# Autodesk Inventor assembly: BrImp_Assembly
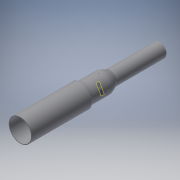
[picture p0: Inventor's stored thumbnail of the model, 180x180]
Saved by Autodesk Inventor 2018 (Build 220112000, 112)
## iProperties
Created: 2018-02-04
Part Number: BrImp_Assembly
Document SubType Name: Assembly
Designer: Benedikt
Author: Benedikt
## Documents named in this file (13)
- E:\3Dprinting\Stuff\Brushlessstuff\BrushlessImpeller\BrImp_Assembly.iam
- E:\3Dprinting\Stuff\Brushlessstuff\BrushlessImpeller\BrImp_Motormodel.ipt
- E:\3Dprinting\Stuff\Brushlessstuff\BrushlessImpeller\BRImp_Mount.ipt
- E:\3Dprinting\Stuff\Brushlessstuff\BrushlessImpeller\BrImp_Bridge.ipt
- E:\3Dprinting\Stuff\Brushlessstuff\BrushlessImpeller\BrImp_Casing_v01.ipt
- E:\3Dprinting\Stuff\Brushlessstuff\BrushlessImpeller\brImp_fan_actual.ipt
- E:\3Dprinting\Stuff\Brushlessstuff\BrushlessImpeller\frontchute.ipt
- E:\3Dprinting\Stuff\Brushlessstuff\BrushlessImpeller\chuteback.ipt
- E:\3Dprinting\Stuff\Brushlessstuff\BrushlessImpeller\rotatingregion.ipt
- E:\3Dprinting\Stuff\Brushlessstuff\BrushlessImpeller\chutecap1.ipt
- E:\3Dprinting\Stuff\Brushlessstuff\BrushlessImpeller\chutecap2.ipt
- E:\3Dprinting\Stuff\Brushlessstuff\BrushlessImpeller\cap1.ipt
- E:\3Dprinting\Stuff\Brushlessstuff\BrushlessImpeller\brImp_fan_actual_v02.ipt
## Components (12 placed, 12 different names)
1. BrImp_Motormodel:1 — Rotational:1, Flush:1, Rigid:1
2. brImp_fan_actual:1 — Rotational:1, Flush:7
3. BRImp_Mount:1 — Flush:1, Flush:2
4. BrImp_Bridge:1 — Flush:2, Flush:3
5. BrImp_Casing_v01:1 — Flush:3, Flush:4, Flush:5, Flush:6, Flush:10
6. frontchute:1 — Flush:4, Flush:8
7. chuteback:1 — Flush:5, Flush:6, Flush:9
8. rotatingregion:1 — Flush:7
9. chutecap1:1 — Flush:8
10. chutecap2:1 — Flush:9
11. cap1:1 — Flush:10
12. brImp_fan_actual_v02:1 — Rigid:1
## Relationships (12: Flush 10, RevoluteJoint 1, WeldJoint 1)
- Rotational:1 [RevoluteJoint]: BrImp_Motormodel:1 ↔ brImp_fan_actual:1
- Flush:1: BrImp_Motormodel:1 ↔ BRImp_Mount:1
- Flush:2: BRImp_Mount:1 ↔ BrImp_Bridge:1
- Flush:3: BrImp_Bridge:1 ↔ BrImp_Casing_v01:1
- Flush:4: BrImp_Casing_v01:1 ↔ frontchute:1
- Flush:5: BrImp_Casing_v01:1 ↔ chuteback:1
- Flush:6: BrImp_Casing_v01:1 ↔ chuteback:1
- Flush:7: brImp_fan_actual:1 ↔ rotatingregion:1
- Flush:8: frontchute:1 ↔ chutecap1:1
- Flush:9: chuteback:1 ↔ chutecap2:1
- Flush:10: BrImp_Casing_v01:1 ↔ cap1:1
- Rigid:1 [WeldJoint]: BrImp_Motormodel:1 ↔ brImp_fan_actual_v02:1
